# Autodesk Inventor assembly: 3SteelSlides
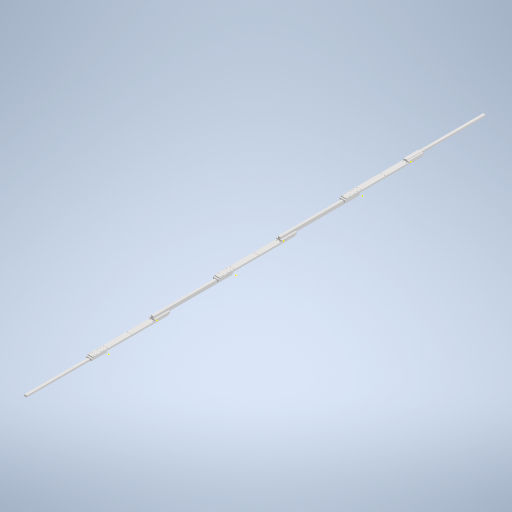
[picture p0: Inventor's stored thumbnail of the model, 512x512]
Saved by Autodesk Inventor 2023 (Build 270158000, 158)
## iProperties
Created: 2022-09-25
Part Number: 3SteelSlides
Document SubType Name: Assembly
Designer: deli
Author: deli
## Documents named in this file (2)
- C:\Users\deli\OneDrive - Eastside Preparatory School\FTC\8103-power-play\CAD\3SteelSlides.iam
- C:\Users\deli\OneDrive - Eastside Preparatory School\FTC\8103-power-play\CAD\steelSlideseExtended.iam
## Components (3 placed, 1 different names)
1. steelSlideseExtended:1 [sub-assembly] — Mate:1, Flush:3, Flush:4
2. steelSlideseExtended:2 [sub-assembly] — Mate:1, Mate:2, Flush:1, Flush:2, Flush:3, Flush:4
3. steelSlideseExtended:3 [sub-assembly] — Mate:2, Flush:1, Flush:2
## Relationships (6: Flush 4, Mate 2)
- Mate:1: steelSlideseExtended:1 ↔ steelSlideseExtended:2
- Mate:2: steelSlideseExtended:2 ↔ steelSlideseExtended:3
- Flush:1: steelSlideseExtended:2 ↔ steelSlideseExtended:3
- Flush:2: steelSlideseExtended:2 ↔ steelSlideseExtended:3
- Flush:3: steelSlideseExtended:1 ↔ steelSlideseExtended:2
- Flush:4: steelSlideseExtended:1 ↔ steelSlideseExtended:2
